# Autodesk Inventor assembly: Zusammenbau
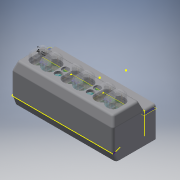
[picture p0: Inventor's stored thumbnail of the model, 180x180]
Saved by Autodesk Inventor 2019 (Build 230136000, 136)
## iProperties
Created: 2019-08-02
Part Number: Zusammenbau
Material: Generisch
Document SubType Name: Assembly
Designer: grubi
Author: grubi
## Documents named in this file (6)
- \\diskstation\home\NixieBaugruppe\Zusammenbau.iam
- \\diskstation\home\NixieBaugruppe\NixieModule_IN12.brd.ipt
- \\diskstation\home\idf\IN-12\IN-12a.ipt
- \\diskstation\home\NixieBaugruppe\Gehaeuse_IN12.ipt
- \\diskstation\home\NixieBaugruppe\NixieMainboard.brd.iam
- \\diskstation\home\NixieBaugruppe\Gehaeuse_IN12_Rueckwand.ipt
## Components (12 placed, 5 different names)
1. Gehaeuse_IN12:1 — Fluchtend:3, Passend:4, Passend:5, Passend:7, Passend:8, Passend:9, Passend:10, Passend:11, Passend:12, Passend:13, Passend:14
2. NixieMainboard.brd:1 [sub-assembly] — Passend:7, Passend:8, Passend:9, Passend:10, Passend:11, Passend:12
3. Gehaeuse_IN12_Rueckwand:1 — Passend:13, Passend:14
4. NixieModule_IN12.brd:1 — Passend:1, Passend:2, Passend:3
5. IN-12a:1 — Fluchtend:1, Fluchtend:2, Passend:1, Passend:3
6. IN-12a:2 — Fluchtend:1, Fluchtend:2, Passend:2
7. NixieModule_IN12.brd:2 — Fluchtend:3, Passend:6
8. IN-12a:3
9. IN-12a:4 — Passend:5
10. NixieModule_IN12.brd:3 — Passend:4
11. IN-12a:5
12. IN-12a:6
## Component patterns: (3 elements, first: NixieModule_IN12.brd:1 + IN-12a:1 + IN-12a:2)
## Relationships (17: Mate 14, Flush 3)
- Fluchtend:1 [Flush]: IN-12a:1 ↔ IN-12a:2
- Fluchtend:2 [Flush]: IN-12a:1 ↔ IN-12a:2
- Passend:1 [Mate] (-34 mm): NixieModule_IN12.brd:1 ↔ IN-12a:1
- Passend:2 [Mate]: NixieModule_IN12.brd:1 ↔ IN-12a:2
- Passend:3 [Mate]: NixieModule_IN12.brd:1 ↔ IN-12a:1
- Fluchtend:3 [Flush]: Gehaeuse_IN12:1 ↔ NixieModule_IN12.brd:2
- Passend:4 [Mate] (14 mm): Gehaeuse_IN12:1 ↔ NixieModule_IN12.brd:3
- Passend:5 [Mate]: Gehaeuse_IN12:1 ↔ IN-12a:4
- Passend:6 [Mate]: NixieModule_IN12.brd:2
- Passend:7 [Mate]: Gehaeuse_IN12:1 ↔ NixieMainboard.brd:1
- Passend:8 [Mate]: Gehaeuse_IN12:1 ↔ NixieMainboard.brd:1
- Passend:9 [Mate]: Gehaeuse_IN12:1 ↔ NixieMainboard.brd:1
- Passend:10 [Mate]: Gehaeuse_IN12:1 ↔ NixieMainboard.brd:1
- Passend:11 [Mate]: Gehaeuse_IN12:1 ↔ NixieMainboard.brd:1
- Passend:12 [Mate]: Gehaeuse_IN12:1 ↔ NixieMainboard.brd:1
- Passend:13 [Mate]: Gehaeuse_IN12:1 ↔ Gehaeuse_IN12_Rueckwand:1
- Passend:14 [Mate]: Gehaeuse_IN12:1 ↔ Gehaeuse_IN12_Rueckwand:1
